# Autodesk Inventor assembly: ChestDerived
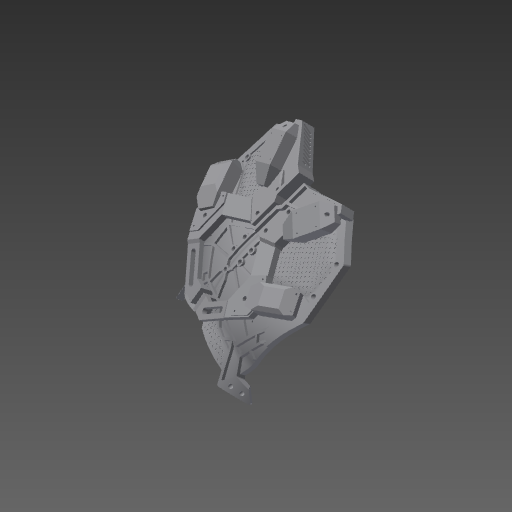
[picture p0: Inventor's stored thumbnail of the model, 512x512]
Saved by Autodesk Inventor 2020 (Build 240168000, 168)
## iProperties
Created: 2015-05-09
Part Number: ChestDerived
Document SubType Name: Assembly
Designer: Val
Author: Val
## Documents named in this file (5)
- C:\Users\valer\Desktop\elysium-max-exoskeleton\src\Assemblies\ChestDerived.iam
- C:\Users\valer\Desktop\elysium-max-exoskeleton\src\ChestBaseDerived.ipt
- C:\Users\valer\Desktop\elysium-max-exoskeleton\src\ChestPlateRightDerived.ipt
- C:\Users\valer\Desktop\elysium-max-exoskeleton\src\ChestPlateLeftDerived.ipt
- C:\Users\valer\Desktop\elysium-max-exoskeleton\src\External\Fan12VDC.ipt
## Components (4 placed, 4 different names)
1. ChestBaseDerived:1 — Mate:1, Mate:2, Flush:1, Flush:2
2. ChestPlateRightDerived:1 — Mate:1, Mate:2, Flush:1, Mate:3
3. ChestPlateLeftDerived:1 — Flush:2
4. Fan12VDC:1 — Mate:3
## Relationships (5: Mate 3, Flush 2)
- Mate:1: ChestBaseDerived:1 ↔ ChestPlateRightDerived:1
- Mate:2: ChestBaseDerived:1 ↔ ChestPlateRightDerived:1
- Flush:1: ChestBaseDerived:1 ↔ ChestPlateRightDerived:1
- Flush:2: ChestBaseDerived:1 ↔ ChestPlateLeftDerived:1
- Mate:3: ChestPlateRightDerived:1 ↔ Fan12VDC:1
